# Autodesk Inventor assembly: Kepala
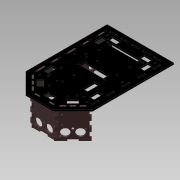
[picture p0: Inventor's stored thumbnail of the model, 180x180]
Saved by Autodesk Inventor 2015 SP1 (Build 190203100, 203)
## iProperties
Created: 2015-02-13
Part Number: Kepala
Document SubType Name: Assembly
Designer: Rafi Kurnia Putra
Author: Rafi Kurnia Putra
## Documents named in this file (6)
- D:\Dropbox\krpai berkaki trui 2015\ROBUSTA\MEKANIK\ROBUSTA\Laser Cutting\Kepala.iam
- D:\Dropbox\krpai berkaki trui 2015\ROBUSTA\MEKANIK\ROBUSTA\Laser Cutting\Base Kepala.ipt
- D:\Dropbox\krpai berkaki trui 2015\ROBUSTA\MEKANIK\ROBUSTA\Laser Cutting\srfdepan.ipt
- D:\Dropbox\krpai berkaki trui 2015\ROBUSTA\MEKANIK\ROBUSTA\Laser Cutting\srfdiagkanan.ipt
- D:\Dropbox\krpai berkaki trui 2015\ROBUSTA\MEKANIK\ROBUSTA\Laser Cutting\srfdiagkiri.ipt
- D:\Dropbox\krpai berkaki trui 2015\ROBUSTA\MEKANIK\ROBUSTA\Laser Cutting\srfsampingkiri.ipt
## Components (5 placed, 5 different names)
1. Base Kepala:1 — Mate:1, Mate:2, Flush:1, Mate:3, Mate:4, Mate:5, Mate:6, Mate:7, Mate:8, Mate:9, Mate:10, Mate:11, Mate:12, Mate:13, Mate:14
2. srfdepan:1 — Mate:3, Mate:4, Mate:5
3. srfdiagkiri:1 — Mate:6, Mate:7, Mate:8
4. srfdiagkanan:1 — Mate:9, Mate:10, Mate:11
5. srfsampingkiri:1 — Mate:12, Mate:13, Mate:14
## Relationships (15: Mate 14, Flush 1)
- Mate:1: Base Kepala:1
- Mate:2: Base Kepala:1
- Flush:1: Base Kepala:1
- Mate:3: Base Kepala:1 ↔ srfdepan:1
- Mate:4: Base Kepala:1 ↔ srfdepan:1
- Mate:5: Base Kepala:1 ↔ srfdepan:1
- Mate:6: Base Kepala:1 ↔ srfdiagkiri:1
- Mate:7: Base Kepala:1 ↔ srfdiagkiri:1
- Mate:8: Base Kepala:1 ↔ srfdiagkiri:1
- Mate:9: Base Kepala:1 ↔ srfdiagkanan:1
- Mate:10: Base Kepala:1 ↔ srfdiagkanan:1
- Mate:11: Base Kepala:1 ↔ srfdiagkanan:1
- Mate:12: Base Kepala:1 ↔ srfsampingkiri:1
- Mate:13: Base Kepala:1 ↔ srfsampingkiri:1
- Mate:14: Base Kepala:1 ↔ srfsampingkiri:1
